# Autodesk Inventor assembly: 付け根_1
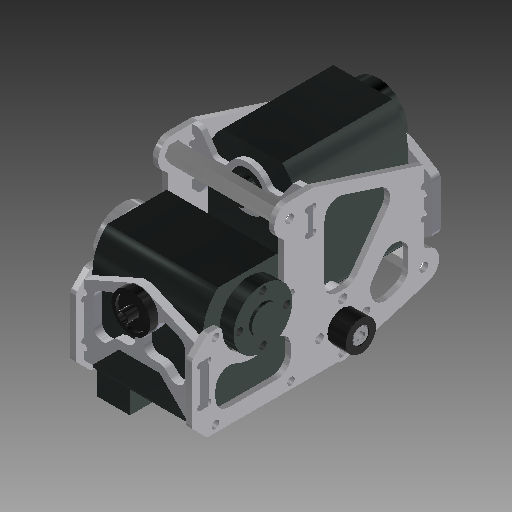
[picture p0: Inventor's stored thumbnail of the model, 512x512]
Saved by Autodesk Inventor 2018 (Build 220112000, 112)
## iProperties
Created: 2016-04-27
Part Number: 付け根_1
Document SubType Name: Assembly
Designer: hiroaki
Mass: 257.123 g
Surface Area: 430.699 cm^2
Volume: 127.027 cm^3
Density: 2.02416 g/cm^3
Author: hiroaki
## Documents named in this file (15)
- C:\Users\taka\Documents\github\OpenPlatform\mechanism\OpenPlatform_ver3_0\下半身_160823\付け根\付け根_1.iam
- C:\Users\taka\Documents\github\OpenPlatform\mechanism\OpenPlatform_ver3_0\既製品\B3M11xx.ipt
- C:\Users\taka\Documents\github\OpenPlatform\mechanism\OpenPlatform_ver3_0\既製品\free_horn.ipt
- C:\Users\taka\Documents\github\OpenPlatform\mechanism\OpenPlatform_ver3_0\下半身_160823\付け根\付け根_サブフレーム_1_2.ipt
- C:\Users\taka\Documents\github\OpenPlatform\mechanism\OpenPlatform_ver3_0\下半身\リンク\スペーサ\付け根_フリー軸_1_1.ipt
- C:\Users\taka\Documents\github\OpenPlatform\mechanism\OpenPlatform_ver3_0\既製品\ASU-340.ipt
- C:\Users\taka\Documents\github\OpenPlatform\mechanism\OpenPlatform_ver3_0\既製品\新規購入\BRU-305_5.ipt
- C:\Users\taka\Documents\github\OpenPlatform\mechanism\OpenPlatform_ver3_0\下半身_160823\付け根\付け根_サブフレーム_6_2.ipt
- C:\Users\taka\Documents\github\OpenPlatform\mechanism\OpenPlatform_ver3_0\下半身_160823\付け根\付け根_サブフレーム_1_4.ipt
- C:\Users\taka\Documents\github\OpenPlatform\mechanism\OpenPlatform_ver3_0\既製品\新規購入\BRU-306_5.ipt
- C:\Users\taka\Documents\github\OpenPlatform\mechanism\OpenPlatform_ver3_0\下半身_160823\付け根\付け根_サブフレーム_6_4.ipt
- C:\Users\taka\Documents\github\OpenPlatform\mechanism\OpenPlatform_ver3_0\下半身_160823\付け根\付け根_メインフレーム_2_1.ipt
- C:\Users\taka\Documents\github\OpenPlatform\mechanism\OpenPlatform_ver3_0\下半身_160823\付け根\付け根_メインフレーム_2_1_MIR.ipt
- C:\Users\taka\Documents\github\OpenPlatform\mechanism\OpenPlatform_ver3_0\下半身_160823\付け根\付け根_サブフレーム_1_3.ipt
- C:\Users\taka\Documents\github\OpenPlatform\mechanism\OpenPlatform_ver3_0\下半身_160823\付け根\付け根_メインフレーム_6_1.ipt
## Components (19 placed, 14 different names)
1. free_horn:1 — 挿入:1
2. B3M11xx:3 — 挿入:1, 挿入:63, 挿入:64, 挿入:67, 挿入:68, メイト:18
3. B3M11xx:4 — 挿入:7, 挿入:8, 挿入:74, 挿入:75
4. 付け根_サブフレーム_1_2:1 — 挿入:7, 挿入:8, メイト:16, フラッシュ:1, 角度:2
5. 付け根_フリー軸_1_1:1 — 挿入:65, 挿入:66
6. 付け根_フリー軸_1_1:2 — 挿入:69, 挿入:70
7. ASU-340:2 — 挿入:72, 角度:1
8. BRU-305_5:1 — 挿入:52, 挿入:76
9. 付け根_サブフレーム_1_4:1 — メイト:17
10. 付け根_サブフレーム_6_2:1 — 挿入:52
11. BRU-306_5:1 — 挿入:55, 挿入:71
12. BRU-306_5:2 — 挿入:58
13. 付け根_サブフレーム_6_4:1 — 挿入:55
14. 付け根_サブフレーム_6_4:2 — 挿入:58
15. 付け根_メインフレーム_2_1:1 — 挿入:63, 挿入:64, 挿入:65, 挿入:66, 挿入:71, 挿入:72, 角度:1, メイト:16, メイト:20, 挿入:73, フラッシュ:1
16. 付け根_メインフレーム_2_1_MIR:1 — 挿入:67, 挿入:68, 挿入:69, 挿入:70, メイト:19
17. 付け根_サブフレーム_1_3:1 — メイト:17, メイト:18, メイト:19, メイト:20
18. ASU-340:3 — 挿入:73, 角度:2
19. 付け根_メインフレーム_6_1:1 — 挿入:74, 挿入:75, 挿入:76
## Relationships (28: Insert 20, Mate 5, Angle 2, Flush 1)
- 挿入:1 [Insert]: free_horn:1 ↔ B3M11xx:3
- 挿入:7 [Insert]: B3M11xx:4 ↔ 付け根_サブフレーム_1_2:1
- 挿入:8 [Insert]: B3M11xx:4 ↔ 付け根_サブフレーム_1_2:1
- 挿入:52 [Insert]: BRU-305_5:1 ↔ 付け根_サブフレーム_6_2:1
- 挿入:55 [Insert]: BRU-306_5:1 ↔ 付け根_サブフレーム_6_4:1
- 挿入:58 [Insert]: BRU-306_5:2 ↔ 付け根_サブフレーム_6_4:2
- 挿入:63 [Insert]: B3M11xx:3 ↔ 付け根_メインフレーム_2_1:1
- 挿入:64 [Insert]: B3M11xx:3 ↔ 付け根_メインフレーム_2_1:1
- 挿入:65 [Insert]: 付け根_フリー軸_1_1:1 ↔ 付け根_メインフレーム_2_1:1
- 挿入:66 [Insert]: 付け根_フリー軸_1_1:1 ↔ 付け根_メインフレーム_2_1:1
- 挿入:67 [Insert]: B3M11xx:3 ↔ 付け根_メインフレーム_2_1_MIR:1
- 挿入:68 [Insert]: B3M11xx:3 ↔ 付け根_メインフレーム_2_1_MIR:1
- 挿入:69 [Insert]: 付け根_フリー軸_1_1:2 ↔ 付け根_メインフレーム_2_1_MIR:1
- 挿入:70 [Insert]: 付け根_フリー軸_1_1:2 ↔ 付け根_メインフレーム_2_1_MIR:1
- 挿入:71 [Insert]: BRU-306_5:1 ↔ 付け根_メインフレーム_2_1:1
- 挿入:72 [Insert]: ASU-340:2 ↔ 付け根_メインフレーム_2_1:1
- 角度:1 [Angle] (0 deg): ASU-340:2 ↔ 付け根_メインフレーム_2_1:1
- メイト:16 [Mate]: 付け根_サブフレーム_1_2:1 ↔ 付け根_メインフレーム_2_1:1
- フラッシュ:1 [Flush]: 付け根_サブフレーム_1_2:1 ↔ 付け根_メインフレーム_2_1:1
- メイト:17 [Mate]: 付け根_サブフレーム_1_4:1 ↔ 付け根_サブフレーム_1_3:1
- メイト:18 [Mate]: B3M11xx:3 ↔ 付け根_サブフレーム_1_3:1
- メイト:19 [Mate]: 付け根_メインフレーム_2_1_MIR:1 ↔ 付け根_サブフレーム_1_3:1
- メイト:20 [Mate] (0.025 mm): 付け根_メインフレーム_2_1:1 ↔ 付け根_サブフレーム_1_3:1
- 挿入:73 [Insert]: 付け根_メインフレーム_2_1:1 ↔ ASU-340:3
- 角度:2 [Angle] (90 deg): 付け根_サブフレーム_1_2:1 ↔ ASU-340:3
- 挿入:74 [Insert]: B3M11xx:4 ↔ 付け根_メインフレーム_6_1:1
- 挿入:75 [Insert]: B3M11xx:4 ↔ 付け根_メインフレーム_6_1:1
- 挿入:76 [Insert]: BRU-305_5:1 ↔ 付け根_メインフレーム_6_1:1
